# Autodesk Inventor assembly: ArmWithGripperAttached
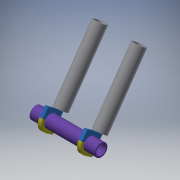
[picture p0: Inventor's stored thumbnail of the model, 180x180]
Saved by Autodesk Inventor 2018.2 (Build 222227000, 227)
## iProperties
Created: 2018-02-13
Part Number: ArmWithGripperAttached
Document SubType Name: Assembly
Designer: steele
Author: steele
## Documents named in this file (4)
- D:\snobotics\CAD-Development\robSteele\2018-FRC\Arm\ArmWithGripperAttached.iam
- D:\snobotics\CAD-Development\robSteele\2018-FRC\Gripper\pipeForExteriorOfGripper.ipt
- D:\snobotics\CAD-Development\robSteele\2018-FRC\Gripper\gripperBracketAssembly.iam
- D:\snobotics\CAD-Development\robSteele\2018-FRC\Arm\endOfArm.ipt
## Components (4 placed, 3 different names)
1. pipeForExteriorOfGripper:1 — Insert:1, Insert:2
2. gripperBracketAssembly:1 [sub-assembly] — Insert:1, Insert:4
3. gripperBracketAssembly:2 [sub-assembly] — Insert:2, Insert:3
4. endOfArm:1 — Insert:3, Insert:4
## Relationships (4: Insert 4)
- Insert:1 (44.45 mm): pipeForExteriorOfGripper:1 ↔ gripperBracketAssembly:1
- Insert:2 (44.45 mm): pipeForExteriorOfGripper:1 ↔ gripperBracketAssembly:2
- Insert:3: gripperBracketAssembly:2 ↔ endOfArm:1
- Insert:4: gripperBracketAssembly:1 ↔ endOfArm:1
